# Autodesk Inventor assembly: CircleFullLegAssembly
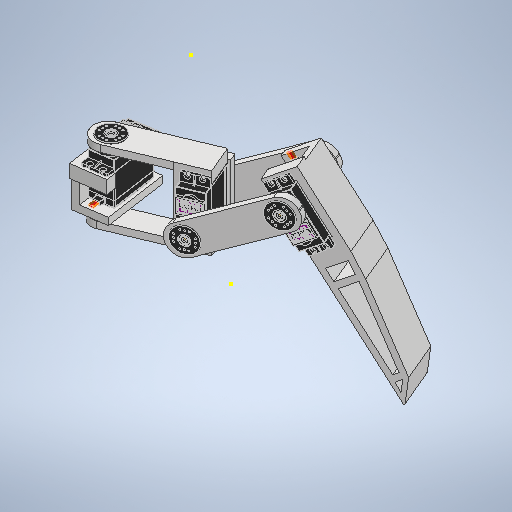
[picture p0: Inventor's stored thumbnail of the model, 512x512]
Saved by Autodesk Inventor 2025.1 (Build 291241020, 241B)
## iProperties
Created: 2024-10-14
Part Number: CircleFullLegAssembly
Document SubType Name: Assembly
Designer: omiye
Author: omiye
## Documents named in this file (7)
- C:\Projects\Arduino\hexapod\legModels\CircleFullLegAssembly.iam
- C:\Projects\Arduino\hexapod\legModels\circleCoxaModel.ipt
- C:\Projects\Arduino\hexapod\legModels\MG996RServoHolder.ipt
- C:\Projects\Arduino\hexapod\legModels\MG996RServo.ipt
- C:\Projects\Arduino\hexapod\legModels\miscStuff\circleServoHorn.ipt
- C:\Projects\Arduino\hexapod\legModels\circleFemurModel.ipt
- C:\Projects\Arduino\hexapod\legModels\tibiaModel.ipt
## Components (10 placed, 6 different names)
1. circleCoxaModel:1 — Mate:6, Mate:7, Mate:8, Mate:9, Mate:10
2. MG996RServoHolder:1 — Mate:3, Mate:4, Mate:5
3. MG996RServo:1 — Mate:1, Mate:2, Mate:3, Mate:4, Mate:5
4. circleServoHorn:1 — Mate:1, Mate:2, Mate:6, Mate:7
5. MG996RServo:2 — Mate:8, Mate:9, Mate:10, Mate:11, Mate:12
6. circleFemurModel:1 — Mate:13, Mate:14, Mate:15, Mate:16
7. circleServoHorn:2 — Mate:11, Mate:12, Mate:13, Mate:14
8. MG996RServo:3 — Mate:17, Mate:18, Mate:19, Mate:20, Mate:21
9. tibiaModel:1 — Mate:19, Mate:20, Mate:21
10. circleServoHorn:3 — Mate:15, Mate:16, Mate:17, Mate:18
## Relationships (21: Mate 21)
- Mate:1: MG996RServo:1 ↔ circleServoHorn:1
- Mate:2: MG996RServo:1 ↔ circleServoHorn:1
- Mate:3: MG996RServoHolder:1 ↔ MG996RServo:1
- Mate:4: MG996RServoHolder:1 ↔ MG996RServo:1
- Mate:5: MG996RServoHolder:1 ↔ MG996RServo:1
- Mate:6: circleCoxaModel:1 ↔ circleServoHorn:1
- Mate:7: circleCoxaModel:1 ↔ circleServoHorn:1
- Mate:8: circleCoxaModel:1 ↔ MG996RServo:2
- Mate:9: circleCoxaModel:1 ↔ MG996RServo:2
- Mate:10: circleCoxaModel:1 ↔ MG996RServo:2
- Mate:11: MG996RServo:2 ↔ circleServoHorn:2
- Mate:12: MG996RServo:2 ↔ circleServoHorn:2
- Mate:13: circleFemurModel:1 ↔ circleServoHorn:2
- Mate:14: circleFemurModel:1 ↔ circleServoHorn:2
- Mate:15: circleFemurModel:1 ↔ circleServoHorn:3
- Mate:16: circleFemurModel:1 ↔ circleServoHorn:3
- Mate:17: MG996RServo:3 ↔ circleServoHorn:3
- Mate:18: MG996RServo:3 ↔ circleServoHorn:3
- Mate:19: MG996RServo:3 ↔ tibiaModel:1
- Mate:20: MG996RServo:3 ↔ tibiaModel:1
- Mate:21: MG996RServo:3 ↔ tibiaModel:1
